# Autodesk Inventor assembly: couple extension arm motor top + pulleys
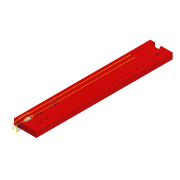
[picture p0: Inventor's stored thumbnail of the model, 180x180]
Saved by Autodesk Inventor 2020 (Build 240168000, 168)
## iProperties
Created: 2019-12-16
Part Number: couple extension arm motor top + pulleys
Document SubType Name: Assembly
Designer: ball
Author: ball
## Documents named in this file (5)
- C:\FTC\FTC8863CAD\2019 Robot\Delivery\extension arm\couple extension arm motor middle + pulleys.iam
- C:\FTC\FTC8863CAD\2019 Robot\Delivery\extension arm\Coupler extension arm motor.ipt
- C:\FTC\FTC8863CAD\2019 Robot\Delivery\plastic pulley deep u.ipt
- C:\FTC\FTC8863CAD\RevRobotics\REV-41-1368 pulley.ipt
- C:\FTC\FTC8863CAD\StepLibraries\Screws\M3 x 20 HEX HEAD CAP SCREW.ipt
## Components (4 placed, 4 different names)
1. Coupler extension arm motor:1 — Mate:5, Mate:6, Mate:7, Mate:8, Mate:9, Mate:10
2. REV-41-1368 pulley:2 — Mate:5, Mate:6
3. plastic pulley deep u:2 — Mate:7, Mate:8
4. M3 x 20 HEX HEAD CAP SCREW:1 — Mate:9, Mate:10
## Relationships (6: Mate 6)
- Mate:5: Coupler extension arm motor:1 ↔ REV-41-1368 pulley:2
- Mate:6: Coupler extension arm motor:1 ↔ REV-41-1368 pulley:2
- Mate:7: Coupler extension arm motor:1 ↔ plastic pulley deep u:2
- Mate:8: Coupler extension arm motor:1 ↔ plastic pulley deep u:2
- Mate:9: Coupler extension arm motor:1 ↔ M3 x 20 HEX HEAD CAP SCREW:1
- Mate:10: Coupler extension arm motor:1 ↔ M3 x 20 HEX HEAD CAP SCREW:1
